# Autodesk Inventor assembly: X-End-Idler v0.1
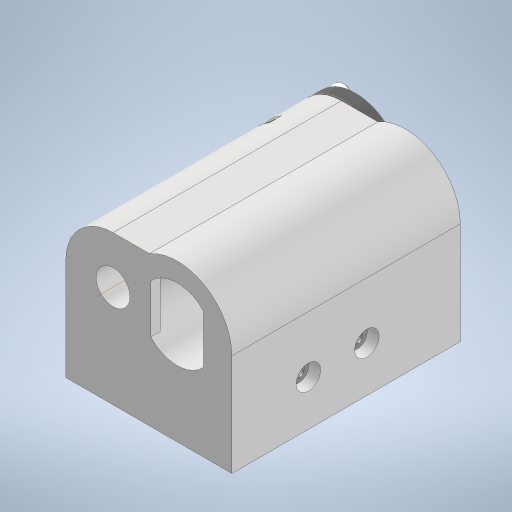
[picture p0: Inventor's stored thumbnail of the model, 512x512]
Saved by Autodesk Inventor 2023 (Build 270158000, 158)
## iProperties
Created: 2023-07-26
Part Number: X-End-Idler v0.1
Document SubType Name: Assembly
Designer: Parker
Author: Parker
## Documents named in this file (10)
- D:\000 - PEPCORP CLOUD\00- Legacy\Designs\MK3PRO P1\X-Axis\X-End-Idler v0.1.iam
- D:\000 - PEPCORP CLOUD\00- Legacy\Designs\MK3PRO P1\X-Axis\X-End-Idler v0.3.ipt
- D:\000 - PEPCORP CLOUD\00- Legacy\Designs\MK3PRO P1\COMPONENTS\Idler Roller, flat.ipt
- D:\000 - PEPCORP CLOUD\00- Legacy\Designs\MK3PRO P1\X-Axis\X-End-Floating-Idler v0.1.ipt
- D:\000 - PEPCORP CLOUD\00- Legacy\Designs\MK3PRO P1\COMPONENTS\SHCS_M5_25.ipt
- D:\000 - PEPCORP CLOUD\00- Legacy\Designs\MK3PRO P1\COMPONENTS\SHCS_M3_25.ipt
- D:\000 - PEPCORP CLOUD\00- Legacy\Designs\MK3PRO P1\COMPONENTS\M5 Nylock.ipt
- D:\000 - PEPCORP CLOUD\00- Legacy\Designs\MK3PRO P1\X-Axis\Z_NUT_1.ipt
- D:\000 - PEPCORP CLOUD\00- Legacy\Designs\MK3PRO P1\COMPONENTS\NUT_SQUARE_M3.ipt
- D:\000 - PEPCORP CLOUD\00- Legacy\Designs\MK3PRO P1\COMPONENTS\SHCS_M3_18.ipt
## Components (14 placed, 9 different names)
1. X-End-Idler v0.3:1 — Mate:1, Mate:2, Mate:3, Mate:4, Mate:5, Mate:6, Mate:7, Mate:15, Mate:16, Mate:21, Mate:22, Angle:3, Angle:4, Mate:23, Mate:24, Mate:25, Mate:26
2. Idler Roller, flat:1 — Mate:8, Mate:9
3. X-End-Floating-Idler v0.1:1 — Mate:1, Mate:2, Mate:3, Mate:8, Mate:9, Mate:12, Mate:13, Mate:14, Mate:17, Mate:18, Mate:19, Mate:20, Angle:1, Angle:2
4. SHCS_M3_25:1 — Mate:4, Mate:7
5. SHCS_M3_25:2 — Mate:5, Mate:6
6. M5 Nylock:1 — Mate:12
7. SHCS_M5_25:1 — Mate:13, Mate:14
8. Z_NUT_1:1 — Mate:23, Mate:24, Mate:25, Mate:26, Mate:27, Mate:28, Mate:29, Mate:30
9. NUT_SQUARE_M3:1 — Mate:17, Mate:20, Angle:1
10. NUT_SQUARE_M3:2 — Mate:16, Mate:21, Angle:4
11. NUT_SQUARE_M3:3 — Mate:18, Mate:19, Angle:2
12. NUT_SQUARE_M3:4 — Mate:15, Mate:22, Angle:3
13. SHCS_M3_18:1 — Mate:28, Mate:29
14. SHCS_M3_18:2 — Mate:27, Mate:30
## Relationships (32: Mate 28, Angle 4)
- Mate:1 (1 mm): X-End-Idler v0.3:1 ↔ X-End-Floating-Idler v0.1:1
- Mate:2: X-End-Idler v0.3:1 ↔ X-End-Floating-Idler v0.1:1
- Mate:3: X-End-Idler v0.3:1 ↔ X-End-Floating-Idler v0.1:1
- Mate:4: X-End-Idler v0.3:1 ↔ SHCS_M3_25:1
- Mate:5: X-End-Idler v0.3:1 ↔ SHCS_M3_25:2
- Mate:6: X-End-Idler v0.3:1 ↔ SHCS_M3_25:2
- Mate:7: X-End-Idler v0.3:1 ↔ SHCS_M3_25:1
- Mate:8: Idler Roller, flat:1 ↔ X-End-Floating-Idler v0.1:1
- Mate:9: Idler Roller, flat:1 ↔ X-End-Floating-Idler v0.1:1
- Mate:12: X-End-Floating-Idler v0.1:1 ↔ M5 Nylock:1
- Mate:13: X-End-Floating-Idler v0.1:1 ↔ SHCS_M5_25:1
- Mate:14: X-End-Floating-Idler v0.1:1 ↔ SHCS_M5_25:1
- Mate:15: X-End-Idler v0.3:1 ↔ NUT_SQUARE_M3:4
- Mate:16: X-End-Idler v0.3:1 ↔ NUT_SQUARE_M3:2
- Mate:17: X-End-Floating-Idler v0.1:1 ↔ NUT_SQUARE_M3:1
- Mate:18: X-End-Floating-Idler v0.1:1 ↔ NUT_SQUARE_M3:3
- Mate:19: X-End-Floating-Idler v0.1:1 ↔ NUT_SQUARE_M3:3
- Mate:20: X-End-Floating-Idler v0.1:1 ↔ NUT_SQUARE_M3:1
- Angle:1 (0 deg): X-End-Floating-Idler v0.1:1 ↔ NUT_SQUARE_M3:1
- Angle:2 (0 deg): X-End-Floating-Idler v0.1:1 ↔ NUT_SQUARE_M3:3
- Mate:21: X-End-Idler v0.3:1 ↔ NUT_SQUARE_M3:2
- Mate:22: X-End-Idler v0.3:1 ↔ NUT_SQUARE_M3:4
- Angle:3 (0 deg): X-End-Idler v0.3:1 ↔ NUT_SQUARE_M3:4
- Angle:4 (0 deg): X-End-Idler v0.3:1 ↔ NUT_SQUARE_M3:2
- Mate:23: X-End-Idler v0.3:1 ↔ Z_NUT_1:1
- Mate:24: X-End-Idler v0.3:1 ↔ Z_NUT_1:1
- Mate:25: X-End-Idler v0.3:1 ↔ Z_NUT_1:1
- Mate:26: X-End-Idler v0.3:1 ↔ Z_NUT_1:1
- Mate:27: Z_NUT_1:1 ↔ SHCS_M3_18:2
- Mate:28: Z_NUT_1:1 ↔ SHCS_M3_18:1
- Mate:29: Z_NUT_1:1 ↔ SHCS_M3_18:1
- Mate:30: Z_NUT_1:1 ↔ SHCS_M3_18:2
